# Autodesk Inventor assembly: zespul12_2
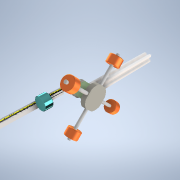
[picture p0: Inventor's stored thumbnail of the model, 180x180]
Saved by Autodesk Inventor 2021 (Build 250183000, 183)
## iProperties
Created: 2021-06-18
Part Number: zespul12_2
Document SubType Name: Assembly
Designer: Wojciech Wołczek
Author: Wojciech Wołczek
## Documents named in this file (8)
- D:\OneDrive\Documents\studia\I rok\labolatoria pracowni fizycznej\pracownia fizyczna 2021 xD\cw 12\zespul12_2.iam
- D:\OneDrive\Documents\studia\I rok\labolatoria pracowni fizycznej\pracownia fizyczna 2021 xD\cw 12\wysiegnik2.ipt
- D:\OneDrive\Documents\studia\I rok\labolatoria pracowni fizycznej\pracownia fizyczna 2021 xD\cw 12\jakis_modulxD.ipt
- D:\OneDrive\Documents\studia\I rok\labolatoria pracowni fizycznej\pracownia fizyczna 2021 xD\cw 12\shaft.ipt
- D:\OneDrive\Documents\studia\I rok\labolatoria pracowni fizycznej\pracownia fizyczna 2021 xD\cw 12\ryrka2.ipt
- D:\OneDrive\Documents\studia\I rok\labolatoria pracowni fizycznej\pracownia fizyczna 2021 xD\cw 12\ciezarek1.ipt
- D:\OneDrive\Documents\studia\I rok\labolatoria pracowni fizycznej\pracownia fizyczna 2021 xD\cw 12\szunr1.ipt
- D:\OneDrive\Documents\studia\I rok\labolatoria pracowni fizycznej\pracownia fizyczna 2021 xD\cw 12\liniau.ipt
## Components (12 placed, 7 different names)
1. wysiegnik2:1 — Zestawiające:4, Zestawiające:5, Równoległe:1, Kątowe:1
2. jakis_modulxD:1 — Zestawiające:1, Zestawiające:2, Zestawiające:3, Równoległe:1, Zestawiające:6, Zestawiające:7
3. shaft:1 — Zestawiające:6, Zestawiające:7, Równoległe:2, Równoległe:3, Kątowe:1, Równoległe:4
4. szunr1:1 — Równoległe:5, Równoległe:6, Równoległe:8, Zestawiające:8, Równoległe:9
5. ciezarek1:5 — Zestawiające:8, Równoległe:9
6. liniau:1 — Równoległe:11, Równoległe:12
7. ryrka2:1 — Równoległe:2, Równoległe:3, Wstawiające:1
8. ryrka2:2
9. ciezarek1:1 — Wstawiające:1
10. ciezarek1:2
11. ciezarek1:3
12. ciezarek1:4
## Component patterns: (2 elements, first: ryrka2:1), (4 elements, first: ciezarek1:1)
## Relationships (22: Flush 12, Mate 8, Insert 1, Angle 1)
- Zestawiające:1 [Mate] (40 mm): jakis_modulxD:1
- Zestawiające:2 [Mate]: jakis_modulxD:1
- Zestawiające:3 [Mate]: jakis_modulxD:1
- Zestawiające:4 [Mate]: wysiegnik2:1
- Zestawiające:5 [Mate]: wysiegnik2:1
- Równoległe:1 [Flush]: wysiegnik2:1 ↔ jakis_modulxD:1
- Zestawiające:6 [Mate]: jakis_modulxD:1 ↔ shaft:1
- Zestawiające:7 [Mate]: jakis_modulxD:1 ↔ shaft:1
- Równoległe:2 [Flush]: shaft:1 ↔ ryrka2:1
- Równoległe:3 [Flush]: shaft:1 ↔ ryrka2:1
- Wstawiające:1 [Insert] (-60 mm): ryrka2:1 ↔ ciezarek1:1
- Kątowe:1 [Angle] (45 deg): wysiegnik2:1 ↔ shaft:1
- Równoległe:4 [Flush] (-10 mm): shaft:1
- Równoległe:5 [Flush]: szunr1:1
- Równoległe:6 [Flush]: szunr1:1
- Równoległe:7 [Flush] (-200 mm)
- Równoległe:8 [Flush]: szunr1:1
- Zestawiające:8 [Mate]: szunr1:1 ↔ ciezarek1:5
- Równoległe:9 [Flush]: szunr1:1 ↔ ciezarek1:5
- Równoległe:10 [Flush] (-100 mm)
- Równoległe:11 [Flush]: liniau:1
- Równoległe:12 [Flush]: liniau:1
